# Autodesk Inventor assembly: Frame
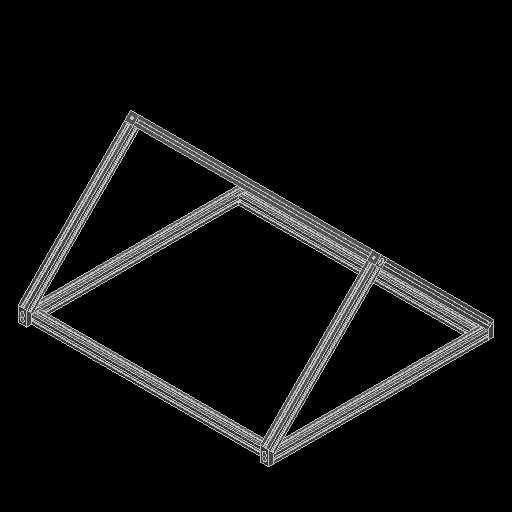
[picture p0: Inventor's stored thumbnail of the model, 512x512]
Saved by Autodesk Inventor 2023 (Build 270158000, 158)
## iProperties
Created: 2023-08-09
Part Number: Frame
Document SubType Name: Assembly
Designer: tandu
Author: tandu
Revision Number: ANY
## Documents named in this file (6)
- C:\Users\tandu\Documents\GrabCAD\Custom Conveyor Belt 3D Printer\V1\Parts\Frame.iam
- C:\Users\tandu\Documents\GrabCAD\Custom Conveyor Belt 3D Printer\V1\Parts\500mm_extrusion.ipt
- C:\Users\tandu\Documents\GrabCAD\Custom Conveyor Belt 3D Printer\V1\Parts\350mm_extrusion.ipt
- C:\Users\tandu\Documents\GrabCAD\Custom Conveyor Belt 3D Printer\V1\Parts\cube.ipt
- C:\Users\tandu\Documents\GrabCAD\Custom Conveyor Belt 3D Printer\V1\Parts\angle_corner_connector_large.ipt
- C:\Users\tandu\Documents\GrabCAD\Custom Conveyor Belt 3D Printer\V1\Parts\Custom_extrusion.ipt
## Components (15 placed, 15 different names)
1. 500mm_extrusion_333 — Insert:1, Flush:1, Insert:5, Flush:5, Mate:1, Flush:6, Flush:7, Mate:3, Flush:10, Flush:11
2. 500mm_extrusion_334 — Flush:8, Mate:2, Flush:9, Insert:7, Insert:8, Flush:15, Flush:16
3. 350mm_extrusion_335 — Insert:9, Flush:13
4. 350mm_extrusion_336 — Insert:4, Flush:4
5. 350mm_extrusion_337 — Insert:2, Flush:2, Insert:3, Flush:3
6. 350mm_extrusion_338 — Insert:10, Insert:11, Flush:14, Flush:17
7. cube_339 — Insert:3, Flush:3, Insert:4, Flush:4, Insert:6, Flush:12, Symmetry:1
8. cube_340 — Insert:11, Flush:17, Symmetry:1
9. 350mm_extrusion_341 — Insert:6, Flush:12
10. 350mm_extrusion_342 — Mate:3, Flush:10, Flush:11
11. 350mm_extrusion_343 — Mate:1, Flush:6, Flush:7, Flush:8, Mate:2, Flush:9
12. angle_corner_connector_large_344 — Insert:1, Flush:1, Insert:2, Flush:2
13. angle_corner_connector_large_345 — Insert:7, Insert:10, Flush:14, Flush:15
14. angle_corner_connector_large_346 — Insert:5, Flush:5
15. angle_corner_connector_large_347 — Insert:8, Insert:9, Flush:13, Flush:16
## Relationships (32: Flush 17, Insert 11, Mate 3, Symmetry 1)
- Insert:1: 500mm_extrusion_333 ↔ angle_corner_connector_large_344
- Flush:1: 500mm_extrusion_333 ↔ angle_corner_connector_large_344
- Insert:2: 350mm_extrusion_337 ↔ angle_corner_connector_large_344
- Flush:2: 350mm_extrusion_337 ↔ angle_corner_connector_large_344
- Insert:3: 350mm_extrusion_337 ↔ cube_339
- Flush:3: 350mm_extrusion_337 ↔ cube_339
- Insert:4: 350mm_extrusion_336 ↔ cube_339
- Flush:4: 350mm_extrusion_336 ↔ cube_339
- Insert:5: 500mm_extrusion_333 ↔ angle_corner_connector_large_346
- Flush:5: 500mm_extrusion_333 ↔ angle_corner_connector_large_346
- Mate:1: 500mm_extrusion_333 ↔ 350mm_extrusion_343
- Flush:6: 500mm_extrusion_333 ↔ 350mm_extrusion_343
- Flush:7: 500mm_extrusion_333 ↔ 350mm_extrusion_343
- Flush:8: 500mm_extrusion_334 ↔ 350mm_extrusion_343
- Mate:2: 500mm_extrusion_334 ↔ 350mm_extrusion_343
- Flush:9: 500mm_extrusion_334 ↔ 350mm_extrusion_343
- Mate:3: 500mm_extrusion_333 ↔ 350mm_extrusion_342
- Flush:10: 500mm_extrusion_333 ↔ 350mm_extrusion_342
- Flush:11: 500mm_extrusion_333 ↔ 350mm_extrusion_342
- Insert:6: cube_339 ↔ 350mm_extrusion_341
- Flush:12: cube_339 ↔ 350mm_extrusion_341
- Insert:7: 500mm_extrusion_334 ↔ angle_corner_connector_large_345
- Insert:8: 500mm_extrusion_334 ↔ angle_corner_connector_large_347
- Insert:9: 350mm_extrusion_335 ↔ angle_corner_connector_large_347
- Insert:10: 350mm_extrusion_338 ↔ angle_corner_connector_large_345
- Insert:11: 350mm_extrusion_338 ↔ cube_340
- Flush:13: 350mm_extrusion_335 ↔ angle_corner_connector_large_347
- Flush:14: 350mm_extrusion_338 ↔ angle_corner_connector_large_345
- Flush:15: 500mm_extrusion_334 ↔ angle_corner_connector_large_345
- Flush:16: 500mm_extrusion_334 ↔ angle_corner_connector_large_347
- Flush:17: 350mm_extrusion_338 ↔ cube_340
- Symmetry:1: cube_339 ↔ cube_340
